(part 1 of 2)
# Autodesk Inventor assembly: deployer assy
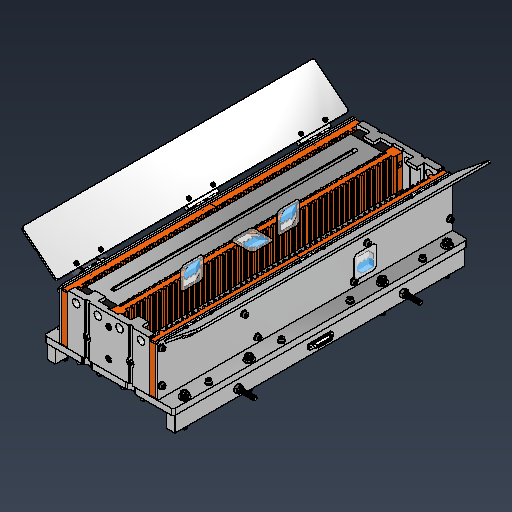
[picture p0: Inventor's stored thumbnail of the model, 512x512]
Saved by Autodesk Inventor 2026.1 (Build 301233000, 233)
## iProperties
Created: 2025-07-24
Part Number: deployer assy
Document SubType Name: Assembly
Designer: richa
Mass: 10916.8 g
Surface Area: 20768.2 cm^2
Volume: 3908.8 cm^3
Density: 2.79287 g/cm^3
Author: richa
## Documents named in this file (37)
- C:\Users\richa\OneDrive\Documents\SSDS\Deployer CAD Files\deployer assy.iam
- C:\Users\richa\OneDrive\Documents\SSDS\Deployer CAD Files\deployer master.ipt
- C:\Users\richa\OneDrive\Documents\SSDS\Deployer CAD Files\base plate.ipt
- C:\Users\richa\OneDrive\Documents\SSDS\Deployer CAD Files\front rack.ipt
- C:\Users\richa\OneDrive\Documents\SSDS\Deployer CAD Files\hull end.ipt
- C:\Users\richa\OneDrive\Documents\SSDS\Deployer CAD Files\launch bar.ipt
- C:\Users\richa\OneDrive\Documents\SSDS\Deployer CAD Files\mid rack.ipt
- C:\Users\richa\OneDrive\Documents\SSDS\Deployer CAD Files\side plate.ipt
- C:\Users\richa\OneDrive\Documents\SSDS\Deployer CAD Files\slider.ipt
- C:\Users\richa\OneDrive\Documents\SSDS\Deployer CAD Files\stilt connector B.ipt
- C:\Users\richa\OneDrive\Documents\SSDS\Deployer CAD Files\stilt connector F.ipt
- C:\Users\richa\OneDrive\Documents\SSDS\Deployer CAD Files\stopper.ipt
- C:\Users\richa\OneDrive\Documents\SSDS\Deployer CAD Files\lid.ipt
- C:\Users\richa\OneDrive\Documents\SSDS\Deployer CAD Files\hinge mount.ipt
- C:\Users\richa\OneDrive\Documents\SSDS\Deployer CAD Files\deployer hardware\93475A230 M4 Stainless Steel Washer.ipt
- C:\Users\richa\OneDrive\Documents\SSDS\Deployer CAD Files\deployer hardware\90576A103_Medium-Strength Steel Nylon-Insert Locknut.ipt
- C:\Users\richa\OneDrive\Documents\SSDS\Deployer CAD Files\deployer hardware\91292A806_22mm 18-8 Stainless Steel Socket Head Screw.ipt
- C:\Users\richa\OneDrive\Documents\SSDS\Deployer CAD Files\deployer hardware\91292A043_18mm 18-8 Stainless Steel Socket Head Screw.ipt
- C:\Users\richa\OneDrive\Documents\SSDS\Deployer CAD Files\deployer hardware\bot leaf.ipt
- C:\Users\richa\OneDrive\Documents\SSDS\Deployer CAD Files\deployer hardware\top leaf.ipt
- C:\Users\richa\OneDrive\Documents\SSDS\Deployer CAD Files\deployer hardware\92855A310_10mm M3 LP 18-8 Stainless Steel Low-Profile Socket Head Screws.ipt
- C:\Users\richa\OneDrive\Documents\SSDS\Deployer CAD Files\V2.3SB\V2.3SB.iam
- C:\Users\richa\OneDrive\Documents\SSDS\Deployer CAD Files\deployer hardware\90576A115 M6 Locknut.ipt
- C:\Users\richa\OneDrive\Documents\SSDS\Deployer CAD Files\deployer hardware\91292A038 14mm M4 Socket Head Screw.ipt
- C:\Users\richa\OneDrive\Documents\SSDS\Deployer CAD Files\deployer hardware\94180A353 7.9mm M4 Brass Tapered Heat-Set.ipt
- C:\Users\richa\OneDrive\Documents\SSDS\Deployer CAD Files\deployer hardware\PC156-1687-6750-MW-3000-CG-N-IN L.ipt
- C:\Users\richa\OneDrive\Documents\SSDS\Deployer CAD Files\deployer hardware\PC156-1687-6750-MW-3000-CG-N-IN S.ipt
- C:\Users\richa\OneDrive\Documents\SSDS\Deployer CAD Files\deployer hardware\90145A484 .156dia .375 long 18-8 Stainless Steel Dowel Pin.ipt
- C:\Users\richa\OneDrive\Documents\SSDS\Deployer CAD Files\deployer hardware\2434K836 70mm M6 Rod End Bolt.ipt
- C:\Users\richa\OneDrive\Documents\SSDS\Deployer CAD Files\deployer hardware\97355A318 40mm 6mm Pull-Out Dowel Pin.ipt
- C:\Users\richa\OneDrive\Documents\SSDS\Deployer CAD Files\deployer hardware\95221A105 M4 Spring Lock Washer.ipt
- C:\Users\richa\OneDrive\Documents\SSDS\Deployer CAD Files\deployer hardware\91235A211 .25in Belleville Spring Lock Washer.ipt
- C:\Users\richa\OneDrive\Documents\SSDS\Deployer CAD Files\deployer hardware\95966A543 1.75in .25-20 Captive Screw.ipt
- C:\Users\richa\OneDrive\Documents\SSDS\Deployer CAD Files\front rack 2.ipt
- C:\Users\richa\OneDrive\Documents\SSDS\Deployer CAD Files\mid rack 2.ipt
- C:\Users\richa\OneDrive\Documents\SSDS\Deployer CAD Files\V2.3.1SB\V2.3.1SB.iam
- C:\Users\richa\OneDrive\Documents\SSDS\Deployer CAD Files\M83513_03-F03N.ipt
## Components (447 placed, 36 different names)
1. deployer master:1 — Flush:1, Flush:2, Flush:3, Rigid:1
2. base plate:1 — Rigid:1, Rigid:2, Rigid:6, Rigid:7, Rigid:9, Cylindrical:2, Angle:1, Cylindrical:3, Angle:2, Rigid:13, Rigid:14, Rigid:17, Rigid:18, Rigid:65, Rigid:67, Rigid:69, Rigid:70, Rigid:80, Rigid:81, Rigid:82, Rigid:83, Rigid:84, Rigid:85, Rigid:86, Rigid:87, Rigid:310, Rigid:311, Rigid:312, Rigid:313, Mate:13, Mate:14, Mate:15, Mate:16, Mate:17, Mate:18, Angle:8, Angle:9, Mate:19, Mate:20, Angle:10, Angle:11, Rigid:336, Rigid:337, Rigid:338, Rigid:339, Rigid:340, Rigid:341, Rigid:342, Rigid:343, Rigid:344, Rigid:345, Rigid:346, Rigid:347, Rigid:3, Rigid:15, Rigid:376, Rigid:377, Rigid:378, Rigid:379, Rigid:380, Rigid:381, Rigid:382, Rigid:383, Rigid:384, Rigid:385, Rigid:386, Rigid:387, Mate:25, Mate:26, Angle:14, Mate:27, Angle:15, Mate:28
3. hull end:1 — Rigid:2, Rigid:4, bars at top, Rigid:321, Rigid:323
4. hull end:2 — Rigid:14, Rigid:318, Rigid:320
5. launch bar:1 — Rigid:8, Cylindrical:2, Angle:1, bars flush, Rigid:10, Mate:29, Flush:12
6. launch bar:2 — Rigid:11, Rigid:12, Cylindrical:3, Angle:2, bars flush, Mate:11, bar at bottom, Flush:10, Mate:23, Flush:11
7. front rack:1 — Rigid:3, Rigid:5, Rigid:133, Rotational:7, Rigid:299, Rigid:356, Rigid:369, Rigid:375
8. front rack:2 — Rigid:15, Rigid:16, Rigid:128, Rigid:300, Rigid:358, Rigid:370, Rigid:371
9. mid rack:1 — Rigid:4, Rigid:41, Rigid:43, Rigid:131, Mate:12, Rigid:368, Rigid:374, Mate:24
10. front rack 2:1 — Rigid:370, Rigid:359, Rigid:301, Rigid:130, Rigid:394, Mate:30
11. front rack 2:2 — Rigid:369, Rigid:132, Rigid:298, Rigid:357, Rigid:373
12. mid rack 2:1 — Rigid:368, Rigid:129, Rigid:55, Rigid:53, Rigid:372
13. side plate:1 — Rigid:5, Rigid:96, Rigid:98, Rigid:99, Rigid:101, Rigid:165, Rigid:166, Rigid:167, lid, Rigid:306, Rigid:307, Rigid:360, Rigid:361
14. side plate:2 — Rigid:16, Rigid:108, Rigid:110, Rigid:111, Rigid:113, Rigid:162, Rigid:163, Rigid:164, Rigid:302, Rigid:303, Rigid:362, Rigid:363
15. stilt connector B:1 — Rigid:7, Rigid:272, Rigid:273, Cylindrical:4, Cylindrical:5
16. stilt connector F:1 — Rigid:6, Rigid:274, Rigid:275, Cylindrical:6, Cylindrical:7, Rigid:395
17. slider:1 — Rigid:8, bars at top, Rigid:252, Rigid:253
18. slider:2 — Rigid:12, Rigid:254, Rigid:255
19. slider:3 — Rigid:11, Rigid:256, Rigid:257
20. slider:4 — Rigid:10, Rigid:258, Rigid:259
21. lid:1 — Rigid:30, Rigid:31, Rigid:32, lid closed, lid up, Rigid:334, Rigid:335, Rigid:332, Rigid:333, Rigid:330, Rigid:331
22. lid:2 — Rigid:33, Rigid:34, Rigid:35, lid closed, lid up, Rigid:324, Rigid:329, Rigid:328, Rigid:327, Rigid:326, Rigid:325
23. stopper:1 — Rigid:9, Rigid:295
24. stopper:2 — Rigid:13, bar at bottom, Rigid:297
25. stopper:3 — Rigid:18, Rigid:296
26. stopper:4 — Rigid:17, Rigid:294
27. M83513_03-F03N:1 — Rigid:395
28. PC156-1687-6750-MW-3000-CG-N-IN L:1 — Mate:15, Mate:19, Angle:10
29. PC156-1687-6750-MW-3000-CG-N-IN L:2 — Mate:16, Mate:20, Angle:11
30. PC156-1687-6750-MW-3000-CG-N-IN L:3 — Mate:27, Angle:15, Mate:28
31. PC156-1687-6750-MW-3000-CG-N-IN S:1 — Mate:14, Mate:18, Angle:9
32. PC156-1687-6750-MW-3000-CG-N-IN S:2 — Mate:13, Mate:17, Angle:8
33. PC156-1687-6750-MW-3000-CG-N-IN S:3 — Mate:25, Mate:26, Angle:14
34. bot leaf:1 — Rigid:165, Rotational:2, Rigid:192, Rigid:193
35. bot leaf:2 — Rigid:166, Rotational:1, Rigid:190, Rigid:191
36. bot leaf:3 — Rigid:167, Rotational:3, Rigid:188, Rigid:189
37. bot leaf:4 — Rigid:162, Rotational:4, Rigid:182, Rigid:183
38. bot leaf:5 — Rigid:163, Rotational:5, Rigid:184, Rigid:185
39. bot leaf:6 — Rigid:164, Rotational:6, Rigid:186, Rigid:187
40. top leaf:1 — Rotational:5, Flush:7, Rigid:290, Rigid:291
41. top leaf:2 — Rotational:4, Flush:8, Rigid:288, Rigid:289
42. top leaf:3 — Rotational:6, Flush:7, Flush:8, Symmetry:1, Rigid:169, Rigid:292, Rigid:293
43. top leaf:4 — Rotational:3, Flush:6, Rigid:282, Rigid:283
44. top leaf:5 — Rotational:2, Flush:5, Flush:6, Symmetry:1, Rigid:168, Rigid:286, Rigid:287
45. top leaf:6 — Rotational:1, Flush:5, Rigid:284, Rigid:285
46. hinge mount:1 — Rigid:34
47. hinge mount:2 — Rigid:33, Rigid:169
48. hinge mount:3 — Rigid:30, Rigid:168, lid
49. hinge mount:4 — Rigid:35
50. hinge mount:5 — Rigid:32
51. hinge mount:6 — Rigid:31
52. 95966A543 1.75in .25-20 Captive Screw:3 — Rigid:354
53. 95966A543 1.75in .25-20 Captive Screw:6 — Rigid:349
54. 95966A543 1.75in .25-20 Captive Screw:5 — Rigid:348
55. 95966A543 1.75in .25-20 Captive Screw:7 — Rigid:350
56. 95966A543 1.75in .25-20 Captive Screw:4 — Rigid:355
57. 95966A543 1.75in .25-20 Captive Screw:8 — Rigid:351
58. 95966A543 1.75in .25-20 Captive Screw:1 — Rigid:352
59. 95966A543 1.75in .25-20 Captive Screw:2 — Rigid:353
60. 91292A043_18mm 18-8 Stainless Steel Socket Head Screw:43 — Rigid:393
61. 91292A043_18mm 18-8 Stainless Steel Socket Head Screw:44 — Rigid:392
62. 91292A043_18mm 18-8 Stainless Steel Socket Head Screw:45 — Rigid:391
63. 91292A043_18mm 18-8 Stainless Steel Socket Head Screw:46 — Rigid:390
64. 91292A043_18mm 18-8 Stainless Steel Socket Head Screw:47 — Rigid:389
65. 91292A043_18mm 18-8 Stainless Steel Socket Head Screw:48 — Rigid:388
66. 91292A038 14mm M4 Socket Head Screw:11 — Rigid:365
67. 91292A038 14mm M4 Socket Head Screw:12 — Rigid:364
68. 91292A038 14mm M4 Socket Head Screw:13 — Rigid:366
69. 91292A038 14mm M4 Socket Head Screw:14 — Rigid:367
70. 91292A043_18mm 18-8 Stainless Steel Socket Head Screw:36
71. 91292A043_18mm 18-8 Stainless Steel Socket Head Screw:37
72. 91292A043_18mm 18-8 Stainless Steel Socket Head Screw:42
73. 91292A043_18mm 18-8 Stainless Steel Socket Head Screw:40
74. 91292A038 14mm M4 Socket Head Screw:7 — Rigid:294
75. 91292A038 14mm M4 Socket Head Screw:8 — Rigid:296
76. 91292A038 14mm M4 Socket Head Screw:9 — Rigid:297
77. 91292A038 14mm M4 Socket Head Screw:10 — Rigid:295
78. 91292A038 14mm M4 Socket Head Screw:2 — Rigid:321
79. 91292A038 14mm M4 Socket Head Screw:3 — Rigid:320
80. 91292A038 14mm M4 Socket Head Screw:5 — Rigid:318
81. 91292A038 14mm M4 Socket Head Screw:6 — Rigid:323
82. 91292A043_18mm 18-8 Stainless Steel Socket Head Screw:13 — Rigid:218
83. 91292A043_18mm 18-8 Stainless Steel Socket Head Screw:14 — Rigid:220
84. 91292A043_18mm 18-8 Stainless Steel Socket Head Screw:15 — Rigid:223
85. 91292A043_18mm 18-8 Stainless Steel Socket Head Screw:16 — Rigid:222
86. 91292A043_18mm 18-8 Stainless Steel Socket Head Screw:17 — Rigid:219
87. 91292A043_18mm 18-8 Stainless Steel Socket Head Screw:18 — Rigid:221
88. 91292A043_18mm 18-8 Stainless Steel Socket Head Screw:38
89. 91292A043_18mm 18-8 Stainless Steel Socket Head Screw:35
90. 91292A043_18mm 18-8 Stainless Steel Socket Head Screw:39
91. 91292A043_18mm 18-8 Stainless Steel Socket Head Screw:41
92. 91292A043_18mm 18-8 Stainless Steel Socket Head Screw:34
93. 91292A043_18mm 18-8 Stainless Steel Socket Head Screw:33
94. 91292A043_18mm 18-8 Stainless Steel Socket Head Screw:32
95. 91292A043_18mm 18-8 Stainless Steel Socket Head Screw:31
96. 91292A043_18mm 18-8 Stainless Steel Socket Head Screw:26
97. 91292A043_18mm 18-8 Stainless Steel Socket Head Screw:25
98. 91292A043_18mm 18-8 Stainless Steel Socket Head Screw:28
99. 91292A043_18mm 18-8 Stainless Steel Socket Head Screw:27
100. 91292A043_18mm 18-8 Stainless Steel Socket Head Screw:22 — Rigid:252
101. 91292A043_18mm 18-8 Stainless Steel Socket Head Screw:29 — Rigid:257
102. 91292A043_18mm 18-8 Stainless Steel Socket Head Screw:20 — Rigid:254
103. 91292A043_18mm 18-8 Stainless Steel Socket Head Screw:21 — Rigid:253
104. 91292A043_18mm 18-8 Stainless Steel Socket Head Screw:19 — Rigid:255
105. 91292A043_18mm 18-8 Stainless Steel Socket Head Screw:23 — Rigid:259
106. 91292A043_18mm 18-8 Stainless Steel Socket Head Screw:24 — Rigid:258
107. 91292A043_18mm 18-8 Stainless Steel Socket Head Screw:30 — Rigid:256
108. 91292A806_22mm 18-8 Stainless Steel Socket Head Screw:36
109. 91292A806_22mm 18-8 Stainless Steel Socket Head Screw:35
110. 91292A806_22mm 18-8 Stainless Steel Socket Head Screw:38
111. 91292A806_22mm 18-8 Stainless Steel Socket Head Screw:37
112. 91292A806_22mm 18-8 Stainless Steel Socket Head Screw:33 — Rigid:117
113. 91292A806_22mm 18-8 Stainless Steel Socket Head Screw:34
114. 91292A806_22mm 18-8 Stainless Steel Socket Head Screw:40
115. 91292A806_22mm 18-8 Stainless Steel Socket Head Screw:39
116. 91292A806_22mm 18-8 Stainless Steel Socket Head Screw:29
117. 91292A806_22mm 18-8 Stainless Steel Socket Head Screw:30
118. 91292A806_22mm 18-8 Stainless Steel Socket Head Screw:31
119. 91292A806_22mm 18-8 Stainless Steel Socket Head Screw:32
120. 93475A230 M4 Stainless Steel Washer:59 — Rigid:379, Rigid:220
121. 93475A230 M4 Stainless Steel Washer:60 — Rigid:382, Rigid:223
122. 93475A230 M4 Stainless Steel Washer:61 — Rigid:378, Rigid:392
123. 93475A230 M4 Stainless Steel Washer:62 — Rigid:380, Rigid:393
124. 93475A230 M4 Stainless Steel Washer:63 — Rigid:381, Rigid:222
125. 93475A230 M4 Stainless Steel Washer:64 — Rigid:383, Rigid:221
126. 93475A230 M4 Stainless Steel Washer:65 — Rigid:384, Rigid:218
127. 93475A230 M4 Stainless Steel Washer:66 — Rigid:385, Rigid:388
128. 93475A230 M4 Stainless Steel Washer:67 — Rigid:386, Rigid:389
129. 93475A230 M4 Stainless Steel Washer:68 — Rigid:387, Rigid:390
130. 93475A230 M4 Stainless Steel Washer:69 — Rigid:377, Rigid:219
131. 93475A230 M4 Stainless Steel Washer:70 — Rigid:376, Rigid:391
132. 93475A230 M4 Stainless Steel Washer:55 — Rigid:360, Rigid:364
133. 93475A230 M4 Stainless Steel Washer:56 — Rigid:361, Rigid:367
134. 93475A230 M4 Stainless Steel Washer:57 — Rigid:362, Rigid:365
135. 93475A230 M4 Stainless Steel Washer:58 — Rigid:363, Rigid:366
136. 95221A105 M4 Spring Lock Washer:8 — Rigid:313
137. 95221A105 M4 Spring Lock Washer:6 — Rigid:312
138. 95221A105 M4 Spring Lock Washer:3 — Rigid:311
139. 95221A105 M4 Spring Lock Washer:2 — Rigid:310
140. 93475A230 M4 Stainless Steel Washer:29 — Rigid:111, Rigid:117
141. 93475A230 M4 Stainless Steel Washer:31 — Rigid:113
142. 93475A230 M4 Stainless Steel Washer:32 — Rigid:108
143. 93475A230 M4 Stainless Steel Washer:34 — Rigid:110
144. 93475A230 M4 Stainless Steel Washer:23 — Rigid:99
145. 93475A230 M4 Stainless Steel Washer:25 — Rigid:101
146. 93475A230 M4 Stainless Steel Washer:26 — Rigid:96
147. 93475A230 M4 Stainless Steel Washer:28 — Rigid:98
148. 95221A105 M4 Spring Lock Washer:17 — Rigid:84
149. 95221A105 M4 Spring Lock Washer:18 — Rigid:85
150. 95221A105 M4 Spring Lock Washer:19 — Rigid:86
151. 95221A105 M4 Spring Lock Washer:20 — Rigid:87
152. 95221A105 M4 Spring Lock Washer:21 — Rigid:80
153. 95221A105 M4 Spring Lock Washer:22 — Rigid:81
154. 95221A105 M4 Spring Lock Washer:23 — Rigid:82
155. 95221A105 M4 Spring Lock Washer:24 — Rigid:83
156. 95221A105 M4 Spring Lock Washer:1 — Rigid:69
157. 95221A105 M4 Spring Lock Washer:4 — Rigid:70
158. 95221A105 M4 Spring Lock Washer:7 — Rigid:67
159. 95221A105 M4 Spring Lock Washer:5 — Rigid:65
160. 93475A230 M4 Stainless Steel Washer:1 — Rigid:303
161. 93475A230 M4 Stainless Steel Washer:2 — Rigid:306
162. 93475A230 M4 Stainless Steel Washer:3 — Rigid:302
163. 93475A230 M4 Stainless Steel Washer:4 — Rigid:307
164. 91235A211 .25in Belleville Spring Lock Washer:1 — Rigid:340, Rigid:352
165. 91235A211 .25in Belleville Spring Lock Washer:2 — Rigid:341, Rigid:353
166. 91235A211 .25in Belleville Spring Lock Washer:6 — Rigid:346, Rigid:349
167. 91235A211 .25in Belleville Spring Lock Washer:3 — Rigid:342, Rigid:354
168. 91235A211 .25in Belleville Spring Lock Washer:7 — Rigid:345, Rigid:350
169. 91235A211 .25in Belleville Spring Lock Washer:5 — Rigid:347, Rigid:348
170. 91235A211 .25in Belleville Spring Lock Washer:4 — Rigid:343, Rigid:355
171. 91235A211 .25in Belleville Spring Lock Washer:8 — Rigid:344, Rigid:351
172. 90576A103_Medium-Strength Steel Nylon-Insert Locknut:1 — Rigid:53
173. 90576A103_Medium-Strength Steel Nylon-Insert Locknut:2 — Rigid:55
174. 90576A103_Medium-Strength Steel Nylon-Insert Locknut:4 — Rigid:43
175. 90576A103_Medium-Strength Steel Nylon-Insert Locknut:6 — Rigid:41
176. 94180A353 7.9mm M4 Brass Tapered Heat-Set:15 — Rigid:374
177. 94180A353 7.9mm M4 Brass Tapered Heat-Set:16 — Rigid:372
178. 94180A353 7.9mm M4 Brass Tapered Heat-Set:17 — Rigid:371
179. 94180A353 7.9mm M4 Brass Tapered Heat-Set:18 — Rigid:373
180. 94180A353 7.9mm M4 Brass Tapered Heat-Set:19 — Rigid:394
181. 94180A353 7.9mm M4 Brass Tapered Heat-Set:20 — Rigid:375
182. 94180A353 7.9mm M4 Brass Tapered Heat-Set:1 — Rigid:301
183. 94180A353 7.9mm M4 Brass Tapered Heat-Set:2 — Rigid:298
184. 94180A353 7.9mm M4 Brass Tapered Heat-Set:3 — Rigid:299
185. 94180A353 7.9mm M4 Brass Tapered Heat-Set:4 — Rigid:300
186. 94180A353 7.9mm M4 Brass Tapered Heat-Set:5 — Rigid:128
187. 94180A353 7.9mm M4 Brass Tapered Heat-Set:6 — Rigid:130
188. 94180A353 7.9mm M4 Brass Tapered Heat-Set:7 — Rigid:131
189. 94180A353 7.9mm M4 Brass Tapered Heat-Set:8 — Rigid:129
190. 94180A353 7.9mm M4 Brass Tapered Heat-Set:9 — Rigid:132
191. 94180A353 7.9mm M4 Brass Tapered Heat-Set:10 — Rigid:133
192. 94180A353 7.9mm M4 Brass Tapered Heat-Set:11 — Rigid:356
193. 94180A353 7.9mm M4 Brass Tapered Heat-Set:12 — Rigid:357
194. 94180A353 7.9mm M4 Brass Tapered Heat-Set:13 — Rigid:358
195. 94180A353 7.9mm M4 Brass Tapered Heat-Set:14 — Rigid:359
196. 92855A310_10mm M3 LP 18-8 Stainless Steel Low-Profile Socket Head Screws:31 — Rigid:329
197. 92855A310_10mm M3 LP 18-8 Stainless Steel Low-Profile Socket Head Screws:32 — Rigid:328
198. 92855A310_10mm M3 LP 18-8 Stainless Steel Low-Profile Socket Head Screws:33 — Rigid:327
199. 92855A310_10mm M3 LP 18-8 Stainless Steel Low-Profile Socket Head Screws:34 — Rigid:326
200. 92855A310_10mm M3 LP 18-8 Stainless Steel Low-Profile Socket Head Screws:35 — Rigid:325
201. 92855A310_10mm M3 LP 18-8 Stainless Steel Low-Profile Socket Head Screws:36 — Rigid:324
202. 92855A310_10mm M3 LP 18-8 Stainless Steel Low-Profile Socket Head Screws:29 — Rigid:334
203. 92855A310_10mm M3 LP 18-8 Stainless Steel Low-Profile Socket Head Screws:30 — Rigid:335
204. 92855A310_10mm M3 LP 18-8 Stainless Steel Low-Profile Socket Head Screws:28 — Rigid:332
205. 92855A310_10mm M3 LP 18-8 Stainless Steel Low-Profile Socket Head Screws:27 — Rigid:333
206. 92855A310_10mm M3 LP 18-8 Stainless Steel Low-Profile Socket Head Screws:25 — Rigid:330
207. 92855A310_10mm M3 LP 18-8 Stainless Steel Low-Profile Socket Head Screws:26 — Rigid:331
208. 92855A310_10mm M3 LP 18-8 Stainless Steel Low-Profile Socket Head Screws:13 — Rigid:289
209. 92855A310_10mm M3 LP 18-8 Stainless Steel Low-Profile Socket Head Screws:14 — Rigid:291
210. 92855A310_10mm M3 LP 18-8 Stainless Steel Low-Profile Socket Head Screws:15 — Rigid:286
211. 92855A310_10mm M3 LP 18-8 Stainless Steel Low-Profile Socket Head Screws:16 — Rigid:282
212. 92855A310_10mm M3 LP 18-8 Stainless Steel Low-Profile Socket Head Screws:17 — Rigid:284
213. 92855A310_10mm M3 LP 18-8 Stainless Steel Low-Profile Socket Head Screws:18 — Rigid:287
214. 92855A310_10mm M3 LP 18-8 Stainless Steel Low-Profile Socket Head Screws:19 — Rigid:290
215. 92855A310_10mm M3 LP 18-8 Stainless Steel Low-Profile Socket Head Screws:20 — Rigid:292
216. 92855A310_10mm M3 LP 18-8 Stainless Steel Low-Profile Socket Head Screws:21 — Rigid:293
217. 92855A310_10mm M3 LP 18-8 Stainless Steel Low-Profile Socket Head Screws:22 — Rigid:288
218. 92855A310_10mm M3 LP 18-8 Stainless Steel Low-Profile Socket Head Screws:23 — Rigid:285
219. 92855A310_10mm M3 LP 18-8 Stainless Steel Low-Profile Socket Head Screws:24 — Rigid:283
220. 92855A310_10mm M3 LP 18-8 Stainless Steel Low-Profile Socket Head Screws:1 — Rigid:182
221. 92855A310_10mm M3 LP 18-8 Stainless Steel Low-Profile Socket Head Screws:2 — Rigid:183
222. 92855A310_10mm M3 LP 18-8 Stainless Steel Low-Profile Socket Head Screws:3 — Rigid:184
223. 92855A310_10mm M3 LP 18-8 Stainless Steel Low-Profile Socket Head Screws:4 — Rigid:185
224. 92855A310_10mm M3 LP 18-8 Stainless Steel Low-Profile Socket Head Screws:5 — Rigid:187
225. 92855A310_10mm M3 LP 18-8 Stainless Steel Low-Profile Socket Head Screws:6 — Rigid:186
226. 92855A310_10mm M3 LP 18-8 Stainless Steel Low-Profile Socket Head Screws:7 — Rigid:188
227. 92855A310_10mm M3 LP 18-8 Stainless Steel Low-Profile Socket Head Screws:8 — Rigid:189
228. 92855A310_10mm M3 LP 18-8 Stainless Steel Low-Profile Socket Head Screws:9 — Rigid:190
229. 92855A310_10mm M3 LP 18-8 Stainless Steel Low-Profile Socket Head Screws:10 — Rigid:191
230. 92855A310_10mm M3 LP 18-8 Stainless Steel Low-Profile Socket Head Screws:11 — Rigid:192
231. 92855A310_10mm M3 LP 18-8 Stainless Steel Low-Profile Socket Head Screws:12 — Rigid:193
232. 97355A318 40mm 6mm Pull-Out Dowel Pin:1
233. 97355A318 40mm 6mm Pull-Out Dowel Pin:2
234. 97355A318 40mm 6mm Pull-Out Dowel Pin:3
235. 97355A318 40mm 6mm Pull-Out Dowel Pin:4
236. 90576A115 M6 Locknut:1 — Rigid:272
237. 90576A115 M6 Locknut:2 — Rigid:273
238. 90576A115 M6 Locknut:3 — Rigid:274
239. 90576A115 M6 Locknut:4 — Rigid:275
240. 2434K836 70mm M6 Rod End Bolt:2 — Cylindrical:5, Mate:21
241. 2434K836 70mm M6 Rod End Bolt:1 — Cylindrical:4, Mate:21, Symmetry:2
242. 2434K836 70mm M6 Rod End Bolt:4 — Cylindrical:6, Mate:22
243. 2434K836 70mm M6 Rod End Bolt:3 — Cylindrical:7, Mate:22, Symmetry:2
244. 90145A484 .156dia .375 long 18-8 Stainless Steel Dowel Pin:1 — Rigid:338
245. 90145A484 .156dia .375 long 18-8 Stainless Steel Dowel Pin:2 — Rigid:339
246. 90145A484 .156dia .375 long 18-8 Stainless Steel Dowel Pin:3 — Rigid:337
247. 90145A484 .156dia .375 long 18-8 Stainless Steel Dowel Pin:4 — Rigid:336
248. V2.3SB:1 [sub-assembly] — Mate:11, Flush:10, Mate:12, Rotational:7
249. V2.3SB:2 [sub-assembly]
250. V2.3SB:3 [sub-assembly]
251. V2.3SB:4 [sub-assembly]
252. V2.3SB:5 [sub-assembly]
253. V2.3SB:6 [sub-assembly]
254. V2.3SB:7 [sub-assembly]
255. V2.3SB:8 [sub-assembly]
256. V2.3SB:9 [sub-assembly]
257. V2.3SB:10 [sub-assembly]
258. V2.3SB:11 [sub-assembly]
259. V2.3SB:12 [sub-assembly]
260. V2.3SB:13 [sub-assembly]
261. V2.3SB:14 [sub-assembly]
262. V2.3SB:15 [sub-assembly]
263. V2.3SB:16 [sub-assembly]
264. V2.3SB:17 [sub-assembly]
265. V2.3SB:18 [sub-assembly]
266. V2.3SB:19 [sub-assembly]
267. V2.3SB:20 [sub-assembly]
268. V2.3SB:21 [sub-assembly]
269. V2.3SB:22 [sub-assembly]
270. V2.3SB:23 [sub-assembly]
271. V2.3SB:24 [sub-assembly]
272. V2.3SB:25 [sub-assembly]
273. V2.3SB:26 [sub-assembly]
274. V2.3SB:27 [sub-assembly]
275. V2.3SB:28 [sub-assembly]
276. V2.3SB:29 [sub-assembly]
277. V2.3SB:30 [sub-assembly]
278. V2.3SB:31 [sub-assembly]
279. V2.3SB:32 [sub-assembly]
280. V2.3SB:33 [sub-assembly]
281. V2.3SB:34 [sub-assembly]
282. V2.3SB:35 [sub-assembly]
283. V2.3SB:36 [sub-assembly]
284. V2.3SB:37 [sub-assembly]
285. V2.3SB:38 [sub-assembly]
286. V2.3SB:39 [sub-assembly]
287. V2.3SB:40 [sub-assembly]
288. V2.3SB:41 [sub-assembly]
289. V2.3SB:42 [sub-assembly]
290. V2.3SB:43 [sub-assembly]
291. V2.3SB:44 [sub-assembly]
292. V2.3SB:45 [sub-assembly]
293. V2.3SB:46 [sub-assembly]
294. V2.3SB:47 [sub-assembly]
295. V2.3SB:48 [sub-assembly]
296. V2.3SB:49 [sub-assembly]
297. V2.3SB:50 [sub-assembly]
298. V2.3SB:51 [sub-assembly]
299. V2.3SB:52 [sub-assembly]
300. V2.3SB:53 [sub-assembly]
301. V2.3SB:54 [sub-assembly]
302. V2.3SB:55 [sub-assembly]
303. V2.3SB:56 [sub-assembly]
304. V2.3SB:57 [sub-assembly]
305. V2.3SB:58 [sub-assembly]
306. V2.3SB:59 [sub-assembly]
307. V2.3SB:60 [sub-assembly]
308. V2.3SB:61 [sub-assembly]
309. V2.3SB:62 [sub-assembly]
310. V2.3SB:63 [sub-assembly]
311. V2.3SB:64 [sub-assembly]
312. V2.3SB:65 [sub-assembly]
313. V2.3SB:66 [sub-assembly]
314. V2.3SB:67 [sub-assembly]
315. V2.3SB:68 [sub-assembly]
316. V2.3SB:69 [sub-assembly]
317. V2.3SB:70 [sub-assembly]
318. V2.3SB:71 [sub-assembly]
319. V2.3SB:72 [sub-assembly]
320. V2.3SB:73 [sub-assembly]
321. V2.3SB:74 [sub-assembly]
322. V2.3SB:75 [sub-assembly]
323. V2.3SB:76 [sub-assembly]
324. V2.3SB:77 [sub-assembly]
325. V2.3SB:78 [sub-assembly]
326. V2.3SB:79 [sub-assembly]
327. V2.3SB:80 [sub-assembly]
328. V2.3SB:81 [sub-assembly]
329. V2.3SB:82 [sub-assembly]
330. V2.3SB:83 [sub-assembly]
331. V2.3SB:84 [sub-assembly]
332. V2.3SB:85 [sub-assembly]
333. V2.3SB:86 [sub-assembly]
334. V2.3SB:87 [sub-assembly]
335. V2.3SB:88 [sub-assembly]
336. V2.3SB:89 [sub-assembly]
337. V2.3SB:90 [sub-assembly]
338. V2.3SB:91 [sub-assembly]
339. V2.3SB:92 [sub-assembly]
340. V2.3SB:93 [sub-assembly]
341. V2.3SB:94 [sub-assembly]
342. V2.3SB:95 [sub-assembly]
343. V2.3SB:96 [sub-assembly]
344. V2.3SB:97 [sub-assembly]
345. V2.3SB:98 [sub-assembly]
346. V2.3SB:99 [sub-assembly]
347. V2.3SB:100 [sub-assembly]
348. V2.3.1SB:1 [sub-assembly] — Mate:23, Flush:11, Mate:24
349. V2.3.1SB:3 [sub-assembly]
350. V2.3.1SB:5 [sub-assembly]
351. V2.3.1SB:7 [sub-assembly]
352. V2.3.1SB:9 [sub-assembly]
353. V2.3.1SB:11 [sub-assembly]
354. V2.3.1SB:13 [sub-assembly]
355. V2.3.1SB:15 [sub-assembly]
356. V2.3.1SB:17 [sub-assembly]
357. V2.3.1SB:19 [sub-assembly]
358. V2.3.1SB:21 [sub-assembly]
359. V2.3.1SB:23 [sub-assembly]
360. V2.3.1SB:25 [sub-assembly]
361. V2.3.1SB:27 [sub-assembly]
362. V2.3.1SB:29 [sub-assembly]
363. V2.3.1SB:31 [sub-assembly]
364. V2.3.1SB:33 [sub-assembly]
365. V2.3.1SB:35 [sub-assembly]
366. V2.3.1SB:37 [sub-assembly]
367. V2.3.1SB:39 [sub-assembly]
368. V2.3.1SB:41 [sub-assembly]
369. V2.3.1SB:43 [sub-assembly]
370. V2.3.1SB:45 [sub-assembly]
371. V2.3.1SB:47 [sub-assembly]
372. V2.3.1SB:49 [sub-assembly]
373. V2.3.1SB:51 [sub-assembly]
374. V2.3.1SB:53 [sub-assembly]
375. V2.3.1SB:55 [sub-assembly]
376. V2.3.1SB:57 [sub-assembly]
377. V2.3.1SB:59 [sub-assembly]
378. V2.3.1SB:61 [sub-assembly]
379. V2.3.1SB:63 [sub-assembly]
380. V2.3.1SB:65 [sub-assembly]
381. V2.3.1SB:67 [sub-assembly]
382. V2.3.1SB:69 [sub-assembly]
383. V2.3.1SB:71 [sub-assembly]
384. V2.3.1SB:73 [sub-assembly]
385. V2.3.1SB:75 [sub-assembly]
386. V2.3.1SB:77 [sub-assembly]
387. V2.3.1SB:79 [sub-assembly]
388. V2.3.1SB:81 [sub-assembly]
389. V2.3.1SB:83 [sub-assembly]
390. V2.3.1SB:85 [sub-assembly]
391. V2.3.1SB:87 [sub-assembly]
392. V2.3.1SB:89 [sub-assembly]
393. V2.3.1SB:91 [sub-assembly]
394. V2.3.1SB:93 [sub-assembly]
395. V2.3.1SB:95 [sub-assembly]
396. V2.3.1SB:97 [sub-assembly]
397. V2.3.1SB:99 [sub-assembly]
398. V2.3.1SB:100 [sub-assembly] — Mate:29, Flush:12, Mate:30
399. V2.3.1SB:101 [sub-assembly]
400. V2.3.1SB:102 [sub-assembly]
401. V2.3.1SB:103 [sub-assembly]
402. V2.3.1SB:104 [sub-assembly]
403. V2.3.1SB:105 [sub-assembly]
404. V2.3.1SB:106 [sub-assembly]
405. V2.3.1SB:107 [sub-assembly]
406. V2.3.1SB:108 [sub-assembly]
407. V2.3.1SB:109 [sub-assembly]
408. V2.3.1SB:110 [sub-assembly]
409. V2.3.1SB:111 [sub-assembly]
410. V2.3.1SB:112 [sub-assembly]
411. V2.3.1SB:113 [sub-assembly]
412. V2.3.1SB:114 [sub-assembly]
413. V2.3.1SB:115 [sub-assembly]
414. V2.3.1SB:116 [sub-assembly]
415. V2.3.1SB:117 [sub-assembly]
416. V2.3.1SB:118 [sub-assembly]
417. V2.3.1SB:119 [sub-assembly]
418. V2.3.1SB:120 [sub-assembly]
419. V2.3.1SB:121 [sub-assembly]
420. V2.3.1SB:122 [sub-assembly]
421. V2.3.1SB:123 [sub-assembly]
422. V2.3.1SB:124 [sub-assembly]
423. V2.3.1SB:125 [sub-assembly]
424. V2.3.1SB:126 [sub-assembly]
425. V2.3.1SB:127 [sub-assembly]
426. V2.3.1SB:128 [sub-assembly]
427. V2.3.1SB:129 [sub-assembly]
428. V2.3.1SB:130 [sub-assembly]
429. V2.3.1SB:131 [sub-assembly]
430. V2.3.1SB:132 [sub-assembly]
431. V2.3.1SB:133 [sub-assembly]
432. V2.3.1SB:134 [sub-assembly]
433. V2.3.1SB:135 [sub-assembly]
434. V2.3.1SB:136 [sub-assembly]
435. V2.3.1SB:137 [sub-assembly]
436. V2.3.1SB:138 [sub-assembly]
437. V2.3.1SB:139 [sub-assembly]
438. V2.3.1SB:140 [sub-assembly]
439. V2.3.1SB:141 [sub-assembly]
440. V2.3.1SB:142 [sub-assembly]
441. V2.3.1SB:143 [sub-assembly]
442. V2.3.1SB:144 [sub-assembly]
443. V2.3.1SB:145 [sub-assembly]
444. V2.3.1SB:146 [sub-assembly]
445. V2.3.1SB:147 [sub-assembly]
446. V2.3.1SB:148 [sub-assembly]
447. V2.3.1SB:149 [sub-assembly]
## Component patterns: (100 elements, first: V2.3SB:1), (50 elements, first: V2.3.1SB:1), (50 elements, first: V2.3.1SB:100)
## Relationships (291: WeldJoint 228, Mate 22, Angle 15, Flush 11, RevoluteJoint 7, CylindricalJoint 6, Symmetry 2)
- lid [Angle] (-51 deg): side plate:1 ↔ hinge mount:3
- lid up [Angle] (0 deg): lid:1 ↔ lid:2
- lid closed [Angle] (0 deg): lid:1 ↔ lid:2
- bar at bottom [Mate]: launch bar:2 ↔ stopper:2
- bars at top [Mate]: hull end:1 ↔ slider:1
- bars flush [Flush]: launch bar:1 ↔ launch bar:2
- Mate:11: launch bar:2 ↔ V2.3SB:1
- Flush:10: launch bar:2 ↔ V2.3SB:1
- Mate:12: mid rack:1 ↔ V2.3SB:1
- Rotational:7 [RevoluteJoint]: front rack:1 ↔ V2.3SB:1
- Flush:1: deployer master:1
- Flush:2: deployer master:1
- Flush:3: deployer master:1
- Symmetry:1: top leaf:3 ↔ top leaf:5
- Rigid:1 [WeldJoint]: deployer master:1 ↔ base plate:1
- Rigid:2 [WeldJoint]: base plate:1 ↔ hull end:1
- Rigid:3 [WeldJoint]: base plate:1 ↔ front rack:1
- Rigid:4 [WeldJoint] (0.127 mm): hull end:1 ↔ mid rack:1
- Rigid:5 [WeldJoint]: front rack:1 ↔ side plate:1
- Rigid:6 [WeldJoint]: base plate:1 ↔ stilt connector F:1
- Rigid:7 [WeldJoint]: base plate:1 ↔ stilt connector B:1
- Rigid:8 [WeldJoint]: launch bar:1 ↔ slider:1
- Rigid:9 [WeldJoint]: base plate:1 ↔ stopper:1
- Cylindrical:2: base plate:1 ↔ launch bar:1
- Angle:1 (0 deg): base plate:1 ↔ launch bar:1
- Rigid:10 [WeldJoint]: launch bar:1 ↔ slider:4
- Rigid:11 [WeldJoint]: launch bar:2 ↔ slider:3
- Rigid:12 [WeldJoint]: launch bar:2 ↔ slider:2
- Cylindrical:3: base plate:1 ↔ launch bar:2
- Angle:2 (0 deg): base plate:1 ↔ launch bar:2
- Rigid:13 [WeldJoint]: base plate:1 ↔ stopper:2
- Rigid:14 [WeldJoint]: base plate:1 ↔ hull end:2
- Rigid:15 [WeldJoint]: base plate:1 ↔ front rack:2
- Rigid:16 [WeldJoint]: front rack:2 ↔ side plate:2
- Rigid:17 [WeldJoint]: base plate:1 ↔ stopper:4
- Rigid:18 [WeldJoint]: base plate:1 ↔ stopper:3
- Rigid:30 [WeldJoint]: lid:1 ↔ hinge mount:3
- Rigid:31 [WeldJoint]: lid:1 ↔ hinge mount:6
- Rigid:32 [WeldJoint]: lid:1 ↔ hinge mount:5
- Rigid:33 [WeldJoint]: lid:2 ↔ hinge mount:2
- Rigid:34 [WeldJoint]: lid:2 ↔ hinge mount:1
- Rigid:35 [WeldJoint]: lid:2 ↔ hinge mount:4
- Rigid:41 [WeldJoint]: mid rack:1 ↔ 90576A103_Medium-Strength Steel Nylon-Insert Locknut:6
- Rigid:43 [WeldJoint]: mid rack:1 ↔ 90576A103_Medium-Strength Steel Nylon-Insert Locknut:4
- Rigid:53 [WeldJoint]: mid rack 2:1 ↔ 90576A103_Medium-Strength Steel Nylon-Insert Locknut:1
- Rigid:55 [WeldJoint]: mid rack 2:1 ↔ 90576A103_Medium-Strength Steel Nylon-Insert Locknut:2
- Rigid:65 [WeldJoint]: base plate:1 ↔ 95221A105 M4 Spring Lock Washer:5
- Rigid:67 [WeldJoint]: base plate:1 ↔ 95221A105 M4 Spring Lock Washer:7
- Rigid:69 [WeldJoint]: base plate:1 ↔ 95221A105 M4 Spring Lock Washer:1
- Rigid:70 [WeldJoint]: base plate:1 ↔ 95221A105 M4 Spring Lock Washer:4
- [WeldJoint]: 91292A043_18mm 18-8 Stainless Steel Socket Head Screw:41 ↔ 95221A105 M4 Spring Lock Washer:7
- [WeldJoint]: 91292A043_18mm 18-8 Stainless Steel Socket Head Screw:39 ↔ 95221A105 M4 Spring Lock Washer:5
- [WeldJoint]: 91292A043_18mm 18-8 Stainless Steel Socket Head Screw:38 ↔ 95221A105 M4 Spring Lock Washer:1
- [WeldJoint]: 91292A043_18mm 18-8 Stainless Steel Socket Head Screw:35 ↔ 95221A105 M4 Spring Lock Washer:4
- Rigid:80 [WeldJoint]: base plate:1 ↔ 95221A105 M4 Spring Lock Washer:21
- Rigid:81 [WeldJoint]: base plate:1 ↔ 95221A105 M4 Spring Lock Washer:22
- Rigid:82 [WeldJoint]: base plate:1 ↔ 95221A105 M4 Spring Lock Washer:23
- Rigid:83 [WeldJoint]: base plate:1 ↔ 95221A105 M4 Spring Lock Washer:24
- Rigid:84 [WeldJoint]: base plate:1 ↔ 95221A105 M4 Spring Lock Washer:17
- Rigid:85 [WeldJoint]: base plate:1 ↔ 95221A105 M4 Spring Lock Washer:18
- Rigid:86 [WeldJoint]: base plate:1 ↔ 95221A105 M4 Spring Lock Washer:19
- Rigid:87 [WeldJoint]: base plate:1 ↔ 95221A105 M4 Spring Lock Washer:20
- [WeldJoint]: 91292A043_18mm 18-8 Stainless Steel Socket Head Screw:26 ↔ 95221A105 M4 Spring Lock Washer:21
- [WeldJoint]: 91292A043_18mm 18-8 Stainless Steel Socket Head Screw:25 ↔ 95221A105 M4 Spring Lock Washer:22
- [WeldJoint]: 91292A043_18mm 18-8 Stainless Steel Socket Head Screw:28 ↔ 95221A105 M4 Spring Lock Washer:23
- [WeldJoint]: 91292A043_18mm 18-8 Stainless Steel Socket Head Screw:27 ↔ 95221A105 M4 Spring Lock Washer:24
- [WeldJoint]: 91292A043_18mm 18-8 Stainless Steel Socket Head Screw:34 ↔ 95221A105 M4 Spring Lock Washer:17
- [WeldJoint]: 91292A043_18mm 18-8 Stainless Steel Socket Head Screw:33 ↔ 95221A105 M4 Spring Lock Washer:18
- [WeldJoint]: 91292A043_18mm 18-8 Stainless Steel Socket Head Screw:32 ↔ 95221A105 M4 Spring Lock Washer:19
- [WeldJoint]: 91292A043_18mm 18-8 Stainless Steel Socket Head Screw:31 ↔ 95221A105 M4 Spring Lock Washer:20
- Rigid:96 [WeldJoint]: side plate:1 ↔ 93475A230 M4 Stainless Steel Washer:26
- Rigid:98 [WeldJoint]: side plate:1 ↔ 93475A230 M4 Stainless Steel Washer:28
- Rigid:99 [WeldJoint]: side plate:1 ↔ 93475A230 M4 Stainless Steel Washer:23
- Rigid:101 [WeldJoint]: side plate:1 ↔ 93475A230 M4 Stainless Steel Washer:25
- [WeldJoint]: 91292A806_22mm 18-8 Stainless Steel Socket Head Screw:38 ↔ 93475A230 M4 Stainless Steel Washer:26
- [WeldJoint]: 91292A806_22mm 18-8 Stainless Steel Socket Head Screw:37 ↔ 93475A230 M4 Stainless Steel Washer:28
- [WeldJoint]: 91292A806_22mm 18-8 Stainless Steel Socket Head Screw:36 ↔ 93475A230 M4 Stainless Steel Washer:23
- [WeldJoint]: 91292A806_22mm 18-8 Stainless Steel Socket Head Screw:35 ↔ 93475A230 M4 Stainless Steel Washer:25
- Rigid:108 [WeldJoint]: side plate:2 ↔ 93475A230 M4 Stainless Steel Washer:32
- Rigid:110 [WeldJoint]: side plate:2 ↔ 93475A230 M4 Stainless Steel Washer:34
- Rigid:111 [WeldJoint]: side plate:2 ↔ 93475A230 M4 Stainless Steel Washer:29
- Rigid:113 [WeldJoint]: side plate:2 ↔ 93475A230 M4 Stainless Steel Washer:31
- [WeldJoint]: 91292A806_22mm 18-8 Stainless Steel Socket Head Screw:40 ↔ 93475A230 M4 Stainless Steel Washer:32
- [WeldJoint]: 91292A806_22mm 18-8 Stainless Steel Socket Head Screw:39 ↔ 93475A230 M4 Stainless Steel Washer:34
- Rigid:117 [WeldJoint]: 91292A806_22mm 18-8 Stainless Steel Socket Head Screw:33 ↔ 93475A230 M4 Stainless Steel Washer:29
- [WeldJoint]: 91292A806_22mm 18-8 Stainless Steel Socket Head Screw:34 ↔ 93475A230 M4 Stainless Steel Washer:31
- Rigid:128 [WeldJoint]: front rack:2 ↔ 94180A353 7.9mm M4 Brass Tapered Heat-Set:5
- Rigid:129 [WeldJoint]: mid rack 2:1 ↔ 94180A353 7.9mm M4 Brass Tapered Heat-Set:8
- Rigid:130 [WeldJoint]: front rack 2:1 ↔ 94180A353 7.9mm M4 Brass Tapered Heat-Set:6
- Rigid:131 [WeldJoint]: mid rack:1 ↔ 94180A353 7.9mm M4 Brass Tapered Heat-Set:7
- Rigid:132 [WeldJoint]: front rack 2:2 ↔ 94180A353 7.9mm M4 Brass Tapered Heat-Set:9
- Rigid:133 [WeldJoint]: front rack:1 ↔ 94180A353 7.9mm M4 Brass Tapered Heat-Set:10
- Rigid:162 [WeldJoint]: side plate:2 ↔ bot leaf:4
- Rigid:163 [WeldJoint]: side plate:2 ↔ bot leaf:5
- Rigid:164 [WeldJoint]: side plate:2 ↔ bot leaf:6
- Rigid:165 [WeldJoint]: side plate:1 ↔ bot leaf:1
- Rigid:166 [WeldJoint]: side plate:1 ↔ bot leaf:2
- Rigid:167 [WeldJoint]: side plate:1 ↔ bot leaf:3
- Rotational:1 [RevoluteJoint]: bot leaf:2 ↔ top leaf:6
- Rotational:2 [RevoluteJoint]: bot leaf:1 ↔ top leaf:5
- Rotational:3 [RevoluteJoint]: bot leaf:3 ↔ top leaf:4
- Rotational:4 [RevoluteJoint]: bot leaf:4 ↔ top leaf:2
- Rotational:5 [RevoluteJoint]: bot leaf:5 ↔ top leaf:1
- Rotational:6 [RevoluteJoint]: bot leaf:6 ↔ top leaf:3
- Flush:5: top leaf:5 ↔ top leaf:6
- Flush:6: top leaf:4 ↔ top leaf:5
- Flush:7: top leaf:1 ↔ top leaf:3
- Flush:8: top leaf:2 ↔ top leaf:3
- Rigid:168 [WeldJoint]: top leaf:5 ↔ hinge mount:3
- Rigid:169 [WeldJoint]: top leaf:3 ↔ hinge mount:2
- Rigid:182 [WeldJoint]: bot leaf:4 ↔ 92855A310_10mm M3 LP 18-8 Stainless Steel Low-Profile Socket Head Screws:1
- Rigid:183 [WeldJoint]: bot leaf:4 ↔ 92855A310_10mm M3 LP 18-8 Stainless Steel Low-Profile Socket Head Screws:2
- Rigid:184 [WeldJoint]: bot leaf:5 ↔ 92855A310_10mm M3 LP 18-8 Stainless Steel Low-Profile Socket Head Screws:3
- Rigid:185 [WeldJoint]: bot leaf:5 ↔ 92855A310_10mm M3 LP 18-8 Stainless Steel Low-Profile Socket Head Screws:4
- Rigid:186 [WeldJoint]: bot leaf:6 ↔ 92855A310_10mm M3 LP 18-8 Stainless Steel Low-Profile Socket Head Screws:6
- Rigid:187 [WeldJoint]: bot leaf:6 ↔ 92855A310_10mm M3 LP 18-8 Stainless Steel Low-Profile Socket Head Screws:5
- Rigid:188 [WeldJoint]: bot leaf:3 ↔ 92855A310_10mm M3 LP 18-8 Stainless Steel Low-Profile Socket Head Screws:7
- Rigid:189 [WeldJoint]: bot leaf:3 ↔ 92855A310_10mm M3 LP 18-8 Stainless Steel Low-Profile Socket Head Screws:8
- Rigid:190 [WeldJoint]: bot leaf:2 ↔ 92855A310_10mm M3 LP 18-8 Stainless Steel Low-Profile Socket Head Screws:9
- Rigid:191 [WeldJoint]: bot leaf:2 ↔ 92855A310_10mm M3 LP 18-8 Stainless Steel Low-Profile Socket Head Screws:10
- Rigid:192 [WeldJoint]: bot leaf:1 ↔ 92855A310_10mm M3 LP 18-8 Stainless Steel Low-Profile Socket Head Screws:11
- Rigid:193 [WeldJoint]: bot leaf:1 ↔ 92855A310_10mm M3 LP 18-8 Stainless Steel Low-Profile Socket Head Screws:12
- Rigid:218 [WeldJoint]: 91292A043_18mm 18-8 Stainless Steel Socket Head Screw:13 ↔ 93475A230 M4 Stainless Steel Washer:65
- Rigid:219 [WeldJoint]: 91292A043_18mm 18-8 Stainless Steel Socket Head Screw:17 ↔ 93475A230 M4 Stainless Steel Washer:69
- Rigid:220 [WeldJoint]: 91292A043_18mm 18-8 Stainless Steel Socket Head Screw:14 ↔ 93475A230 M4 Stainless Steel Washer:59
- Rigid:221 [WeldJoint]: 91292A043_18mm 18-8 Stainless Steel Socket Head Screw:18 ↔ 93475A230 M4 Stainless Steel Washer:64
- Rigid:222 [WeldJoint]: 91292A043_18mm 18-8 Stainless Steel Socket Head Screw:16 ↔ 93475A230 M4 Stainless Steel Washer:63
- Rigid:223 [WeldJoint]: 91292A043_18mm 18-8 Stainless Steel Socket Head Screw:15 ↔ 93475A230 M4 Stainless Steel Washer:60
- [WeldJoint] (4 mm): hull end:1 ↔ 97355A318 40mm 6mm Pull-Out Dowel Pin:1
- [WeldJoint] (4 mm): hull end:1 ↔ 97355A318 40mm 6mm Pull-Out Dowel Pin:4
- [WeldJoint] (4 mm): hull end:2 ↔ 97355A318 40mm 6mm Pull-Out Dowel Pin:3
- [WeldJoint] (4 mm): hull end:2 ↔ 97355A318 40mm 6mm Pull-Out Dowel Pin:2
- Rigid:252 [WeldJoint]: slider:1 ↔ 91292A043_18mm 18-8 Stainless Steel Socket Head Screw:22
- Rigid:253 [WeldJoint]: slider:1 ↔ 91292A043_18mm 18-8 Stainless Steel Socket Head Screw:21
- Rigid:254 [WeldJoint]: slider:2 ↔ 91292A043_18mm 18-8 Stainless Steel Socket Head Screw:20
- Rigid:255 [WeldJoint]: slider:2 ↔ 91292A043_18mm 18-8 Stainless Steel Socket Head Screw:19
- Rigid:256 [WeldJoint]: slider:3 ↔ 91292A043_18mm 18-8 Stainless Steel Socket Head Screw:30
- Rigid:257 [WeldJoint]: slider:3 ↔ 91292A043_18mm 18-8 Stainless Steel Socket Head Screw:29
- Rigid:258 [WeldJoint]: slider:4 ↔ 91292A043_18mm 18-8 Stainless Steel Socket Head Screw:24
- Rigid:259 [WeldJoint]: slider:4 ↔ 91292A043_18mm 18-8 Stainless Steel Socket Head Screw:23
- Rigid:272 [WeldJoint]: stilt connector B:1 ↔ 90576A115 M6 Locknut:1
- Rigid:273 [WeldJoint]: stilt connector B:1 ↔ 90576A115 M6 Locknut:2
- Rigid:274 [WeldJoint]: stilt connector F:1 ↔ 90576A115 M6 Locknut:3
- Rigid:275 [WeldJoint]: stilt connector F:1 ↔ 90576A115 M6 Locknut:4
- Cylindrical:4: stilt connector B:1 ↔ 2434K836 70mm M6 Rod End Bolt:1
- Cylindrical:5: stilt connector B:1 ↔ 2434K836 70mm M6 Rod End Bolt:2
- Cylindrical:6: stilt connector F:1 ↔ 2434K836 70mm M6 Rod End Bolt:4
- Cylindrical:7: stilt connector F:1 ↔ 2434K836 70mm M6 Rod End Bolt:3
- [Angle] (0 deg): base plate:1 ↔ 2434K836 70mm M6 Rod End Bolt:4
- [Angle] (0 deg): base plate:1 ↔ 2434K836 70mm M6 Rod End Bolt:3
- [Angle] (0 deg): base plate:1 ↔ 2434K836 70mm M6 Rod End Bolt:2
- [Angle] (0 deg): base plate:1 ↔ 2434K836 70mm M6 Rod End Bolt:1
- Rigid:282 [WeldJoint]: top leaf:4 ↔ 92855A310_10mm M3 LP 18-8 Stainless Steel Low-Profile Socket Head Screws:16
- Rigid:283 [WeldJoint]: top leaf:4 ↔ 92855A310_10mm M3 LP 18-8 Stainless Steel Low-Profile Socket Head Screws:24
- Rigid:284 [WeldJoint]: top leaf:6 ↔ 92855A310_10mm M3 LP 18-8 Stainless Steel Low-Profile Socket Head Screws:17
- Rigid:285 [WeldJoint]: top leaf:6 ↔ 92855A310_10mm M3 LP 18-8 Stainless Steel Low-Profile Socket Head Screws:23
- Rigid:286 [WeldJoint]: top leaf:5 ↔ 92855A310_10mm M3 LP 18-8 Stainless Steel Low-Profile Socket Head Screws:15
- Rigid:287 [WeldJoint]: top leaf:5 ↔ 92855A310_10mm M3 LP 18-8 Stainless Steel Low-Profile Socket Head Screws:18
- Rigid:288 [WeldJoint]: top leaf:2 ↔ 92855A310_10mm M3 LP 18-8 Stainless Steel Low-Profile Socket Head Screws:22
- Rigid:289 [WeldJoint]: top leaf:2 ↔ 92855A310_10mm M3 LP 18-8 Stainless Steel Low-Profile Socket Head Screws:13
- Rigid:290 [WeldJoint]: top leaf:1 ↔ 92855A310_10mm M3 LP 18-8 Stainless Steel Low-Profile Socket Head Screws:19
- Rigid:291 [WeldJoint]: top leaf:1 ↔ 92855A310_10mm M3 LP 18-8 Stainless Steel Low-Profile Socket Head Screws:14
- Rigid:292 [WeldJoint]: top leaf:3 ↔ 92855A310_10mm M3 LP 18-8 Stainless Steel Low-Profile Socket Head Screws:20
- Rigid:293 [WeldJoint]: top leaf:3 ↔ 92855A310_10mm M3 LP 18-8 Stainless Steel Low-Profile Socket Head Screws:21
- Rigid:294 [WeldJoint]: stopper:4 ↔ 91292A038 14mm M4 Socket Head Screw:7
- Rigid:295 [WeldJoint]: stopper:1 ↔ 91292A038 14mm M4 Socket Head Screw:10
- Rigid:296 [WeldJoint]: stopper:3 ↔ 91292A038 14mm M4 Socket Head Screw:8
- Rigid:297 [WeldJoint]: stopper:2 ↔ 91292A038 14mm M4 Socket Head Screw:9
- Rigid:298 [WeldJoint]: front rack 2:2 ↔ 94180A353 7.9mm M4 Brass Tapered Heat-Set:2
- Rigid:299 [WeldJoint]: front rack:1 ↔ 94180A353 7.9mm M4 Brass Tapered Heat-Set:3
- Rigid:300 [WeldJoint]: front rack:2 ↔ 94180A353 7.9mm M4 Brass Tapered Heat-Set:4
- Rigid:301 [WeldJoint]: front rack 2:1 ↔ 94180A353 7.9mm M4 Brass Tapered Heat-Set:1
- Rigid:302 [WeldJoint]: side plate:2 ↔ 93475A230 M4 Stainless Steel Washer:3
- Rigid:303 [WeldJoint]: side plate:2 ↔ 93475A230 M4 Stainless Steel Washer:1
- [WeldJoint]: 91292A806_22mm 18-8 Stainless Steel Socket Head Screw:30 ↔ 93475A230 M4 Stainless Steel Washer:1
- [WeldJoint]: 91292A806_22mm 18-8 Stainless Steel Socket Head Screw:32 ↔ 93475A230 M4 Stainless Steel Washer:3
- Rigid:306 [WeldJoint]: side plate:1 ↔ 93475A230 M4 Stainless Steel Washer:2
- Rigid:307 [WeldJoint]: side plate:1 ↔ 93475A230 M4 Stainless Steel Washer:4
- [WeldJoint]: 91292A806_22mm 18-8 Stainless Steel Socket Head Screw:29 ↔ 93475A230 M4 Stainless Steel Washer:2
- [WeldJoint]: 91292A806_22mm 18-8 Stainless Steel Socket Head Screw:31 ↔ 93475A230 M4 Stainless Steel Washer:4
- Rigid:310 [WeldJoint]: base plate:1 ↔ 95221A105 M4 Spring Lock Washer:2
- Rigid:311 [WeldJoint]: base plate:1 ↔ 95221A105 M4 Spring Lock Washer:3
- Rigid:312 [WeldJoint]: base plate:1 ↔ 95221A105 M4 Spring Lock Washer:6
- Rigid:313 [WeldJoint]: base plate:1 ↔ 95221A105 M4 Spring Lock Washer:8
- [WeldJoint]: 91292A043_18mm 18-8 Stainless Steel Socket Head Screw:40 ↔ 95221A105 M4 Spring Lock Washer:6
- [WeldJoint]: 91292A043_18mm 18-8 Stainless Steel Socket Head Screw:42 ↔ 95221A105 M4 Spring Lock Washer:8
- [WeldJoint]: 91292A043_18mm 18-8 Stainless Steel Socket Head Screw:36 ↔ 95221A105 M4 Spring Lock Washer:3
- [WeldJoint]: 91292A043_18mm 18-8 Stainless Steel Socket Head Screw:37 ↔ 95221A105 M4 Spring Lock Washer:2
- Rigid:318 [WeldJoint]: hull end:2 ↔ 91292A038 14mm M4 Socket Head Screw:5
- Rigid:320 [WeldJoint]: hull end:2 ↔ 91292A038 14mm M4 Socket Head Screw:3
- Rigid:321 [WeldJoint]: hull end:1 ↔ 91292A038 14mm M4 Socket Head Screw:2
- Rigid:323 [WeldJoint]: hull end:1 ↔ 91292A038 14mm M4 Socket Head Screw:6
- Rigid:324 [WeldJoint]: lid:2 ↔ 92855A310_10mm M3 LP 18-8 Stainless Steel Low-Profile Socket Head Screws:36
- Rigid:325 [WeldJoint]: lid:2 ↔ 92855A310_10mm M3 LP 18-8 Stainless Steel Low-Profile Socket Head Screws:35
- Rigid:326 [WeldJoint]: lid:2 ↔ 92855A310_10mm M3 LP 18-8 Stainless Steel Low-Profile Socket Head Screws:34
- Rigid:327 [WeldJoint]: lid:2 ↔ 92855A310_10mm M3 LP 18-8 Stainless Steel Low-Profile Socket Head Screws:33
- Rigid:328 [WeldJoint]: lid:2 ↔ 92855A310_10mm M3 LP 18-8 Stainless Steel Low-Profile Socket Head Screws:32
- Rigid:329 [WeldJoint]: lid:2 ↔ 92855A310_10mm M3 LP 18-8 Stainless Steel Low-Profile Socket Head Screws:31
- Rigid:330 [WeldJoint]: lid:1 ↔ 92855A310_10mm M3 LP 18-8 Stainless Steel Low-Profile Socket Head Screws:25
- Rigid:331 [WeldJoint]: lid:1 ↔ 92855A310_10mm M3 LP 18-8 Stainless Steel Low-Profile Socket Head Screws:26
- Rigid:332 [WeldJoint]: lid:1 ↔ 92855A310_10mm M3 LP 18-8 Stainless Steel Low-Profile Socket Head Screws:28
- Rigid:333 [WeldJoint]: lid:1 ↔ 92855A310_10mm M3 LP 18-8 Stainless Steel Low-Profile Socket Head Screws:27
- Rigid:334 [WeldJoint]: lid:1 ↔ 92855A310_10mm M3 LP 18-8 Stainless Steel Low-Profile Socket Head Screws:29
- Rigid:335 [WeldJoint]: lid:1 ↔ 92855A310_10mm M3 LP 18-8 Stainless Steel Low-Profile Socket Head Screws:30
- Mate:13: base plate:1 ↔ PC156-1687-6750-MW-3000-CG-N-IN S:2
- Mate:14: base plate:1 ↔ PC156-1687-6750-MW-3000-CG-N-IN S:1
- Mate:15: base plate:1 ↔ PC156-1687-6750-MW-3000-CG-N-IN L:1
- Mate:16: base plate:1 ↔ PC156-1687-6750-MW-3000-CG-N-IN L:2
- Mate:17: base plate:1 ↔ PC156-1687-6750-MW-3000-CG-N-IN S:2
- Mate:18: base plate:1 ↔ PC156-1687-6750-MW-3000-CG-N-IN S:1
- Angle:8 (0 deg): base plate:1 ↔ PC156-1687-6750-MW-3000-CG-N-IN S:2
- Angle:9 (0 deg): base plate:1 ↔ PC156-1687-6750-MW-3000-CG-N-IN S:1
- Mate:19: base plate:1 ↔ PC156-1687-6750-MW-3000-CG-N-IN L:1
- Mate:20: base plate:1 ↔ PC156-1687-6750-MW-3000-CG-N-IN L:2
- Angle:10 (0 deg): base plate:1 ↔ PC156-1687-6750-MW-3000-CG-N-IN L:1
- Angle:11 (0 deg): base plate:1 ↔ PC156-1687-6750-MW-3000-CG-N-IN L:2
- Rigid:336 [WeldJoint]: base plate:1 ↔ 90145A484 .156dia .375 long 18-8 Stainless Steel Dowel Pin:4
- Rigid:337 [WeldJoint]: base plate:1 ↔ 90145A484 .156dia .375 long 18-8 Stainless Steel Dowel Pin:3
- Rigid:338 [WeldJoint]: base plate:1 ↔ 90145A484 .156dia .375 long 18-8 Stainless Steel Dowel Pin:1
- Rigid:339 [WeldJoint]: base plate:1 ↔ 90145A484 .156dia .375 long 18-8 Stainless Steel Dowel Pin:2
- Mate:21: 2434K836 70mm M6 Rod End Bolt:2 ↔ 2434K836 70mm M6 Rod End Bolt:1
- Mate:22: 2434K836 70mm M6 Rod End Bolt:4 ↔ 2434K836 70mm M6 Rod End Bolt:3
- Rigid:340 [WeldJoint]: base plate:1 ↔ 91235A211 .25in Belleville Spring Lock Washer:1
- Rigid:341 [WeldJoint]: base plate:1 ↔ 91235A211 .25in Belleville Spring Lock Washer:2
- Rigid:342 [WeldJoint]: base plate:1 ↔ 91235A211 .25in Belleville Spring Lock Washer:3
- Rigid:343 [WeldJoint]: base plate:1 ↔ 91235A211 .25in Belleville Spring Lock Washer:4
- Rigid:344 [WeldJoint]: base plate:1 ↔ 91235A211 .25in Belleville Spring Lock Washer:8
- Rigid:345 [WeldJoint]: base plate:1 ↔ 91235A211 .25in Belleville Spring Lock Washer:7
- Rigid:346 [WeldJoint]: base plate:1 ↔ 91235A211 .25in Belleville Spring Lock Washer:6
- Rigid:347 [WeldJoint]: base plate:1 ↔ 91235A211 .25in Belleville Spring Lock Washer:5
- Rigid:348 [WeldJoint]: 95966A543 1.75in .25-20 Captive Screw:5 ↔ 91235A211 .25in Belleville Spring Lock Washer:5
- Rigid:349 [WeldJoint]: 95966A543 1.75in .25-20 Captive Screw:6 ↔ 91235A211 .25in Belleville Spring Lock Washer:6
- Rigid:350 [WeldJoint]: 95966A543 1.75in .25-20 Captive Screw:7 ↔ 91235A211 .25in Belleville Spring Lock Washer:7
- Rigid:351 [WeldJoint]: 95966A543 1.75in .25-20 Captive Screw:8 ↔ 91235A211 .25in Belleville Spring Lock Washer:8
- Rigid:352 [WeldJoint]: 95966A543 1.75in .25-20 Captive Screw:1 ↔ 91235A211 .25in Belleville Spring Lock Washer:1
- Rigid:353 [WeldJoint]: 95966A543 1.75in .25-20 Captive Screw:2 ↔ 91235A211 .25in Belleville Spring Lock Washer:2
- Rigid:354 [WeldJoint]: 95966A543 1.75in .25-20 Captive Screw:3 ↔ 91235A211 .25in Belleville Spring Lock Washer:3
- Rigid:355 [WeldJoint]: 95966A543 1.75in .25-20 Captive Screw:4 ↔ 91235A211 .25in Belleville Spring Lock Washer:4
- Rigid:356 [WeldJoint]: front rack:1 ↔ 94180A353 7.9mm M4 Brass Tapered Heat-Set:11
- Rigid:357 [WeldJoint]: front rack 2:2 ↔ 94180A353 7.9mm M4 Brass Tapered Heat-Set:12
- Rigid:358 [WeldJoint]: front rack:2 ↔ 94180A353 7.9mm M4 Brass Tapered Heat-Set:13
- Rigid:359 [WeldJoint]: front rack 2:1 ↔ 94180A353 7.9mm M4 Brass Tapered Heat-Set:14
- Rigid:360 [WeldJoint]: side plate:1 ↔ 93475A230 M4 Stainless Steel Washer:55
- Rigid:361 [WeldJoint]: side plate:1 ↔ 93475A230 M4 Stainless Steel Washer:56
- Rigid:362 [WeldJoint]: side plate:2 ↔ 93475A230 M4 Stainless Steel Washer:57
- Rigid:363 [WeldJoint]: side plate:2 ↔ 93475A230 M4 Stainless Steel Washer:58
- Rigid:364 [WeldJoint]: 91292A038 14mm M4 Socket Head Screw:12 ↔ 93475A230 M4 Stainless Steel Washer:55
- Rigid:365 [WeldJoint]: 91292A038 14mm M4 Socket Head Screw:11 ↔ 93475A230 M4 Stainless Steel Washer:57
- Rigid:366 [WeldJoint]: 91292A038 14mm M4 Socket Head Screw:13 ↔ 93475A230 M4 Stainless Steel Washer:58
- Rigid:367 [WeldJoint]: 91292A038 14mm M4 Socket Head Screw:14 ↔ 93475A230 M4 Stainless Steel Washer:56
- Symmetry:2: 2434K836 70mm M6 Rod End Bolt:1 ↔ 2434K836 70mm M6 Rod End Bolt:3
- Rigid:368 [WeldJoint]: mid rack:1 ↔ mid rack 2:1
- Rigid:369 [WeldJoint]: front rack:1 ↔ front rack 2:2
- Rigid:370 [WeldJoint]: front rack:2 ↔ front rack 2:1
- Rigid:371 [WeldJoint]: front rack:2 ↔ 94180A353 7.9mm M4 Brass Tapered Heat-Set:17
- Rigid:372 [WeldJoint]: mid rack 2:1 ↔ 94180A353 7.9mm M4 Brass Tapered Heat-Set:16
- Rigid:373 [WeldJoint]: front rack 2:2 ↔ 94180A353 7.9mm M4 Brass Tapered Heat-Set:18
- Rigid:394 [WeldJoint]: front rack 2:1 ↔ 94180A353 7.9mm M4 Brass Tapered Heat-Set:19
- Rigid:374 [WeldJoint]: mid rack:1 ↔ 94180A353 7.9mm M4 Brass Tapered Heat-Set:15
- Rigid:375 [WeldJoint]: front rack:1 ↔ 94180A353 7.9mm M4 Brass Tapered Heat-Set:20
- Rigid:376 [WeldJoint]: base plate:1 ↔ 93475A230 M4 Stainless Steel Washer:70
- Rigid:377 [WeldJoint]: base plate:1 ↔ 93475A230 M4 Stainless Steel Washer:69
- Rigid:378 [WeldJoint]: base plate:1 ↔ 93475A230 M4 Stainless Steel Washer:61
- Rigid:379 [WeldJoint]: base plate:1 ↔ 93475A230 M4 Stainless Steel Washer:59
- Rigid:380 [WeldJoint]: base plate:1 ↔ 93475A230 M4 Stainless Steel Washer:62